# Autodesk Inventor assembly: Bloc_moteur
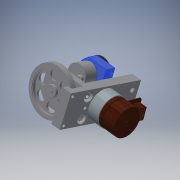
[picture p0: Inventor's stored thumbnail of the model, 180x180]
Saved by Autodesk Inventor 2018 (Build 220112000, 112)
## iProperties
Created: 2019-11-05
Part Number: Bloc_moteur
Document SubType Name: Assembly
Designer: hugo
Author: hugo
## Documents named in this file (23)
- C:\Travail\EIRBOT\Bloc_moteur\Bloc_moteur.iam
- C:\Travail\EIRBOT\Bloc_moteur\Base_moteur.ipt
- C:\Travail\EIRBOT\Bloc_moteur\Base_roue.ipt
- C:\Users\hugo\Documents\Inventor\Content Center Files\R2018\en-US\ANSI B18.3.1M(1)\ANSI B18.3.1M - M6x1 x 20(2).ipt
- C:\Travail\EIRBOT\Bloc_moteur\Bloc_moteur\Design Accelerator\Bearing2.iam
- C:\Travail\EIRBOT\Bloc_moteur\Bloc_moteur\Design Accelerator\Bearing4.iam
- C:\Travail\EIRBOT\Bloc_moteur\301175_GS45A-3st.ipt
- C:\Travail\EIRBOT\Bloc_moteur\397172_EC45fl_70W_A.ipt
- C:\Travail\EIRBOT\Bloc_moteur\Engrenage_spiro_conique.ipt
- C:\Travail\EIRBOT\Bloc_moteur\rondelle.ipt
- C:\Users\hugo\Documents\Inventor\Content Center Files\R2018\en-US\DIN 471(3)\DIN 471 - 8 x 0,8.ipt
- C:\Travail\EIRBOT\Bloc_moteur\tige_roue.ipt
- C:\Travail\EIRBOT\Bloc_moteur\Epaulement_teflon.ipt
- C:\Travail\EIRBOT\Bloc_moteur\Roue.ipt
- C:\Travail\EIRBOT\Bloc_moteur\Codeur_rotatif.ipt
- C:\Travail\EIRBOT\Bloc_moteur\Porte_encodeur.ipt
- C:\Users\hugo\Documents\Inventor\Content Center Files\R2018\en-US\ANSI B18.3.1M(1)\ANSI B18.3.1M - M3x0,5 x 8(2).ipt
- C:\Travail\EIRBOT\Bloc_moteur\Bloc_moteur\Design Accelerator\Shaft1.iam
- C:\Travail\EIRBOT\Bloc_moteur\Roue_encodeuse.ipt
- C:\Travail\EIRBOT\Bloc_moteur\Bloc_moteur\Design Accelerator\Shaft2.iam
- C:\Users\hugo\Documents\Inventor\Content Center Files\R2018\en-US\ANSI B27.7(1)\ANSI B27.7 - 75,55(1).ipt
- C:\Users\hugo\Documents\Inventor\Content Center Files\R2018\en-US\BS 4518(1)\BS 4518 - 0315-30(1).ipt
- C:\Travail\EIRBOT\Bloc_moteur\Bloc_moteur\Design Accelerator\Compress Spring1.iam
## Components (26 placed, 20 different names)
1. Base_moteur:1 — Mate:1, Mate:2, Mate:3, Mate:4, Mate:5, Mate:6, Mate:7, Mate:9, Flush:2, Mate:10, Mate:11, Mate:12, Mate:15, Mate:50, Cylindrical:1
2. Base_roue:1 — Mate:1, Mate:2, Mate:3, Mate:8, Flush:1, Mate:23
3. Broached Socket Head Cap Screw - Metric M6x1 x 20:1 — Mate:6, Mate:7
4. Broached Socket Head Cap Screw - Metric M6x1 x 20:2 — Mate:4, Mate:5
5. Bearing:1 [sub-assembly] — Mate:8, Flush:1, Mate:19, Mate:20, Mate:22, Mate:24
6. Bearing:2 [sub-assembly] — Mate:9, Flush:2
7. 301175_GS45A-3st:1 — Mate:10, Mate:11, Mate:12, Mate:13, Mate:14, Mate:16, Mate:18
8. 397172_EC45fl_70W_A:1 — Mate:13, Mate:14
9. Engrenage_spiro_conique:1 — Mate:17, Mate:18
10. Engrenage_spiro_conique:2 — Mate:21, Mate:22
11. rondelle:1 — Mate:15, Mate:16, Mate:17
12. rondelle:2 — Mate:19, Mate:20, Mate:21
13. DIN 471 <= 9mm 8 x 0,8:1 — Mate:25, Mate:26
14. tige_roue:1 — Mate:25, Mate:26, Mate:27, Mate:28, Mate:29, Mate:30
15. Epaulement_teflon:1 — Mate:23, Mate:24, Mate:27, Mate:28
16. Roue:1 — Mate:29, Mate:30
17. Codeur_rotatif:1 — Mate:31, Mate:32, Mate:33, Mate:40, Mate:41, Mate:42
18. Porte_encodeur:1 — Mate:31, Mate:32, Mate:33, Mate:37, Mate:38, Mate:39, Mate:44, Mate:45, Mate:46, Mate:49, Flush:3
19. Broached Socket Head Cap Screw - Metric M3x0,5 x 8:1 — Mate:37, Mate:38
20. Broached Socket Head Cap Screw - Metric M3x0,5 x 8:2 — Mate:39, Mate:40
21. Shaft:1 [sub-assembly] — Mate:44, Mate:47, Mate:49, Mate:52, Cylindrical:1, Mate:53
22. Roue_encodeuse:1 — Mate:41, Mate:42, Mate:51, Tangent:1
23. Shaft:2 [sub-assembly] — Mate:45, Mate:46, Mate:50
24. E-Ring 7:1 — Mate:47, Mate:52
25. BS 4518 0315-30:1 — Mate:51, Tangent:1
26. Compress Spring:1 [sub-assembly] — Mate:53, Flush:3
## Relationships (53: Mate 48, Flush 3, Tangent 1, CylindricalJoint 1)
- Mate:1: Base_moteur:1 ↔ Base_roue:1
- Mate:2: Base_moteur:1 ↔ Base_roue:1
- Mate:3: Base_moteur:1 ↔ Base_roue:1
- Mate:4: Base_moteur:1 ↔ Broached Socket Head Cap Screw - Metric M6x1 x 20:2
- Mate:5: Base_moteur:1 ↔ Broached Socket Head Cap Screw - Metric M6x1 x 20:2
- Mate:6: Base_moteur:1 ↔ Broached Socket Head Cap Screw - Metric M6x1 x 20:1
- Mate:7: Base_moteur:1 ↔ Broached Socket Head Cap Screw - Metric M6x1 x 20:1
- Mate:8: Base_roue:1 ↔ Bearing:1
- Flush:1: Base_roue:1 ↔ Bearing:1
- Mate:9: Base_moteur:1 ↔ Bearing:2
- Flush:2: Base_moteur:1 ↔ Bearing:2
- Mate:10: Base_moteur:1 ↔ 301175_GS45A-3st:1
- Mate:11: Base_moteur:1 ↔ 301175_GS45A-3st:1
- Mate:12: Base_moteur:1 ↔ 301175_GS45A-3st:1
- Mate:13: 301175_GS45A-3st:1 ↔ 397172_EC45fl_70W_A:1
- Mate:14: 301175_GS45A-3st:1 ↔ 397172_EC45fl_70W_A:1
- Mate:15: Base_moteur:1 ↔ rondelle:1
- Mate:16: 301175_GS45A-3st:1 ↔ rondelle:1
- Mate:17: Engrenage_spiro_conique:1 ↔ rondelle:1
- Mate:18: 301175_GS45A-3st:1 ↔ Engrenage_spiro_conique:1
- Mate:19: Bearing:1 ↔ rondelle:2
- Mate:20: Bearing:1 ↔ rondelle:2
- Mate:21: Engrenage_spiro_conique:2 ↔ rondelle:2
- Mate:22: Bearing:1 ↔ Engrenage_spiro_conique:2
- Mate:23: Base_roue:1 ↔ Epaulement_teflon:1
- Mate:24: Bearing:1 ↔ Epaulement_teflon:1
- Mate:25: DIN 471 <= 9mm 8 x 0,8:1 ↔ tige_roue:1
- Mate:26: DIN 471 <= 9mm 8 x 0,8:1 ↔ tige_roue:1
- Mate:27: tige_roue:1 ↔ Epaulement_teflon:1
- Mate:28: tige_roue:1 ↔ Epaulement_teflon:1
- Mate:29: tige_roue:1 ↔ Roue:1
- Mate:30: tige_roue:1 ↔ Roue:1
- Mate:31: Codeur_rotatif:1 ↔ Porte_encodeur:1
- Mate:32: Codeur_rotatif:1 ↔ Porte_encodeur:1
- Mate:33: Codeur_rotatif:1 ↔ Porte_encodeur:1
- Mate:37: Porte_encodeur:1 ↔ Broached Socket Head Cap Screw - Metric M3x0,5 x 8:1
- Mate:38: Porte_encodeur:1 ↔ Broached Socket Head Cap Screw - Metric M3x0,5 x 8:1
- Mate:39: Porte_encodeur:1 ↔ Broached Socket Head Cap Screw - Metric M3x0,5 x 8:2
- Mate:40: Codeur_rotatif:1 ↔ Broached Socket Head Cap Screw - Metric M3x0,5 x 8:2
- Mate:41: Codeur_rotatif:1 ↔ Roue_encodeuse:1
- Mate:42: Codeur_rotatif:1 ↔ Roue_encodeuse:1
- Mate:44: Porte_encodeur:1 ↔ Shaft:1
- Mate:45: Porte_encodeur:1 ↔ Shaft:2
- Mate:46: Porte_encodeur:1 ↔ Shaft:2
- Mate:47: Shaft:1 ↔ E-Ring 7:1
- Mate:49: Porte_encodeur:1 ↔ Shaft:1
- Mate:50: Base_moteur:1 ↔ Shaft:2
- Mate:51: Roue_encodeuse:1 ↔ BS 4518 0315-30:1
- Tangent:1: Roue_encodeuse:1 ↔ BS 4518 0315-30:1
- Mate:52: Shaft:1 ↔ E-Ring 7:1
- Cylindrical:1: Base_moteur:1 ↔ Shaft:1
- Mate:53: Shaft:1 ↔ Compress Spring:1
- Flush:3: Porte_encodeur:1 ↔ Compress Spring:1
